# Autodesk Inventor assembly: InstrumentAssembly
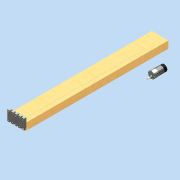
[picture p0: Inventor's stored thumbnail of the model, 180x180]
Saved by Autodesk Inventor 2021 (Build 250183000, 183)
## iProperties
Created: 2021-02-01
Part Number: InstrumentAssembly
Document SubType Name: Assembly
Designer: garre
Author: garre
## Documents named in this file (5)
- C:\Users\garre\Desktop\Parts\InstrumentAssembly.iam
- C:\Users\garre\Desktop\Parts\Body.ipt
- C:\Users\garre\Desktop\Parts\LoadCell.ipt
- C:\Users\garre\Desktop\Parts\Motor.ipt
- C:\Users\garre\Desktop\Parts\String.ipt
## Components (8 placed, 4 different names)
1. Body:1 — Mate:3, Mate:10, Flush:1
2. LoadCell:1 — Mate:9, Flush:5, Flush:9, Insert:1
3. LoadCell:2 — Mate:8, Mate:9, Flush:4, Flush:5, Flush:8
4. LoadCell:3 — Angle:2, Mate:6, Mate:7, Flush:2, Flush:3, Flush:6
5. LoadCell:4 — Mate:7, Mate:8, Flush:3, Flush:4, Flush:7
6. LoadCell:5 — Mate:3, Angle:2, Mate:6, Mate:10, Flush:1, Flush:2, Flush:6, Flush:7, Flush:8, Flush:9
7. Motor:1
8. String:1 — Insert:1
## Relationships (17: Flush 9, Mate 6, Angle 1, Insert 1)
- Mate:3: Body:1 ↔ LoadCell:5
- Angle:2 (0 deg): LoadCell:3 ↔ LoadCell:5
- Mate:6 (19.05 mm): LoadCell:3 ↔ LoadCell:5
- Mate:7 (19.05 mm): LoadCell:3 ↔ LoadCell:4
- Mate:8 (19.05 mm): LoadCell:2 ↔ LoadCell:4
- Mate:9 (19.05 mm): LoadCell:1 ↔ LoadCell:2
- Mate:10 (-31.75 mm): Body:1 ↔ LoadCell:5
- Flush:1: Body:1 ↔ LoadCell:5
- Flush:2: LoadCell:3 ↔ LoadCell:5
- Flush:3: LoadCell:3 ↔ LoadCell:4
- Flush:4: LoadCell:2 ↔ LoadCell:4
- Flush:5: LoadCell:1 ↔ LoadCell:2
- Flush:6: LoadCell:3 ↔ LoadCell:5
- Flush:7: LoadCell:4 ↔ LoadCell:5
- Flush:8: LoadCell:2 ↔ LoadCell:5
- Flush:9: LoadCell:1 ↔ LoadCell:5
- Insert:1: LoadCell:1 ↔ String:1
## Named parameters: stringSeparation = 12.7 mm, loadCellWidth = 12.7 mm, loadCellVerticalOffset = -31.75 mm, loadCellHorizontalOffset = 0 mm, stringLoadCellOffset = 25.4 mm
